# Autodesk Inventor assembly: ThrowerAssemblie
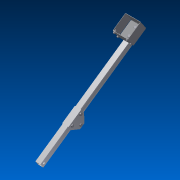
[picture p0: Inventor's stored thumbnail of the model, 180x180]
Saved by Autodesk Inventor 2013 (Build 170138000, 138)
## iProperties
Created: 2013-07-15
Part Number: ThrowerAssemblie
Document SubType Name: Assembly
Designer: root
Author: root
## Documents named in this file (8)
- I:\FRC_Projects\Cad\Inventor_Projects\Shooter-Cleaned\ThrowerAssembly\ThrowerAssemblie.iam
- I:\FRC_Projects\Cad\Inventor_Projects\Shooter-Cleaned\ThrowerAssembly\ArmBAr.ipt
- I:\FRC_Projects\Cad\Inventor_Projects\Shooter-Cleaned\Libraries\ContentCenter\ANSI_ASME B18.2.1 - 1_4-20 UNC - 1.5(2).ipt
- I:\FRC_Projects\Cad\Inventor_Projects\Shooter-Cleaned\Libraries\ContentCenter\AS 2465 - 1_4  UNC(1).ipt
- I:\FRC_Projects\Cad\Inventor_Projects\Shooter-Cleaned\ThrowerAssembly\Mounting.ipt
- I:\FRC_Projects\Cad\Inventor_Projects\Shooter-Cleaned\Libraries\ContentCenter\ANSI B18.2.2 - 1_4 - 20(2).ipt
- I:\FRC_Projects\Cad\Inventor_Projects\Shooter-Cleaned\ThrowerAssembly\Spacer.ipt
- I:\FRC_Projects\Cad\Inventor_Projects\Shooter-Cleaned\ThrowerAssembly\BasketAssembly\NewBasketAssemblie.iam
## Components (16 placed, 7 different names)
1. Hex Bolt - Inch 1/4-20 UNC - 1.5:1 — Mate:21, Mate:23, Mate:45, Mate:49
2. Hex Bolt - Inch 1/4-20 UNC - 1.5:2 — Mate:22, Mate:24, Mate:48
3. AS 2465 - Inch 1/4  UNC:1 — Mate:24, Mate:25
4. AS 2465 - Inch 1/4  UNC:2 — Mate:23, Mate:26
5. ArmBAr:1 — Mate:10, Mate:11, Mate:12, Mate:13, Mate:14, Mate:15, Mate:21, Mate:22, Mate:25, Mate:26, Mate:27, Mate:29, Mate:46, Mate:47
6. Mounting:1 — Mate:10, Mate:14, Mate:15, Mate:28, Mate:30, Mate:36, Mate:37, Mate:41, Mate:42
7. Mounting:2 — Mate:11, Mate:12, Mate:13, Mate:33, Mate:34, Mate:44
8. Hex Bolt - Inch 1/4-20 UNC - 1.5:3 — Mate:27, Mate:28, Mate:32
9. Hex Bolt - Inch 1/4-20 UNC - 1.5:4 — Mate:29, Mate:30, Mate:31
10. Hex Nut - Inch 1/4 - 20:1 — Mate:31, Mate:34
11. Hex Nut - Inch 1/4 - 20:2 — Mate:32, Mate:33
12. Spacer:1 — Mate:36, Mate:37
13. Spacer:2
14. Hex Bolt - Inch 1/4-20 UNC - 1.5:5 — Mate:41, Mate:42, Mate:43
15. Hex Nut - Inch 1/4 - 20:3 — Mate:43, Mate:44
16. NewBasketAssemblie:1 [sub-assembly] — Mate:45, Mate:46, Mate:47, Mate:48, Mate:49
## Relationships (31: Mate 31)
- Mate:10: ArmBAr:1 ↔ Mounting:1
- Mate:11: ArmBAr:1 ↔ Mounting:2
- Mate:12: ArmBAr:1 ↔ Mounting:2
- Mate:13: ArmBAr:1 ↔ Mounting:2
- Mate:14: ArmBAr:1 ↔ Mounting:1
- Mate:15: ArmBAr:1 ↔ Mounting:1
- Mate:21: Hex Bolt - Inch 1/4-20 UNC - 1.5:1 ↔ ArmBAr:1
- Mate:22: Hex Bolt - Inch 1/4-20 UNC - 1.5:2 ↔ ArmBAr:1
- Mate:23: Hex Bolt - Inch 1/4-20 UNC - 1.5:1 ↔ AS 2465 - Inch 1/4  UNC:2
- Mate:24: Hex Bolt - Inch 1/4-20 UNC - 1.5:2 ↔ AS 2465 - Inch 1/4  UNC:1
- Mate:25: AS 2465 - Inch 1/4  UNC:1 ↔ ArmBAr:1
- Mate:26: AS 2465 - Inch 1/4  UNC:2 ↔ ArmBAr:1
- Mate:27: ArmBAr:1 ↔ Hex Bolt - Inch 1/4-20 UNC - 1.5:3
- Mate:28: Mounting:1 ↔ Hex Bolt - Inch 1/4-20 UNC - 1.5:3
- Mate:29: ArmBAr:1 ↔ Hex Bolt - Inch 1/4-20 UNC - 1.5:4
- Mate:30: Mounting:1 ↔ Hex Bolt - Inch 1/4-20 UNC - 1.5:4
- Mate:31: Hex Bolt - Inch 1/4-20 UNC - 1.5:4 ↔ Hex Nut - Inch 1/4 - 20:1
- Mate:32: Hex Bolt - Inch 1/4-20 UNC - 1.5:3 ↔ Hex Nut - Inch 1/4 - 20:2
- Mate:33: Mounting:2 ↔ Hex Nut - Inch 1/4 - 20:2
- Mate:34: Mounting:2 ↔ Hex Nut - Inch 1/4 - 20:1
- Mate:36: Mounting:1 ↔ Spacer:1
- Mate:37: Mounting:1 ↔ Spacer:1
- Mate:41: Mounting:1 ↔ Hex Bolt - Inch 1/4-20 UNC - 1.5:5
- Mate:42: Mounting:1 ↔ Hex Bolt - Inch 1/4-20 UNC - 1.5:5
- Mate:43: Hex Bolt - Inch 1/4-20 UNC - 1.5:5 ↔ Hex Nut - Inch 1/4 - 20:3
- Mate:44: Mounting:2 ↔ Hex Nut - Inch 1/4 - 20:3
- Mate:45: Hex Bolt - Inch 1/4-20 UNC - 1.5:1 ↔ NewBasketAssemblie:1
- Mate:46: ArmBAr:1 ↔ NewBasketAssemblie:1
- Mate:47: ArmBAr:1 ↔ NewBasketAssemblie:1
- Mate:48: Hex Bolt - Inch 1/4-20 UNC - 1.5:2 ↔ NewBasketAssemblie:1
- Mate:49: Hex Bolt - Inch 1/4-20 UNC - 1.5:1 ↔ NewBasketAssemblie:1
